# Autodesk Inventor assembly: Goniometers_70x70
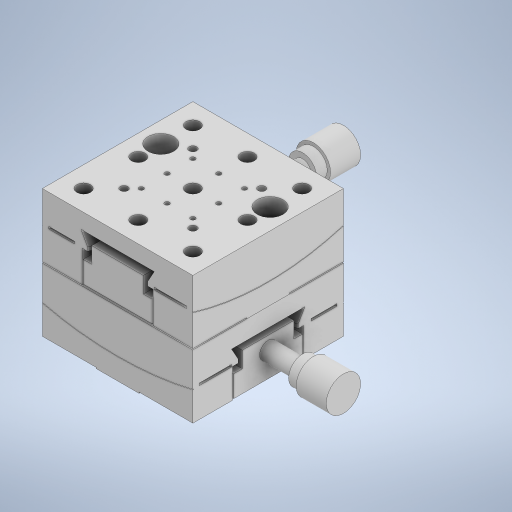
[picture p0: Inventor's stored thumbnail of the model, 512x512]
Saved by Autodesk Inventor 2024 (Build 280153000, 153)
## iProperties
Created: 2022-01-28
Part Number: Goniometers_70x70
Document SubType Name: Assembly
Designer: gnzak
Author: gnzak
## Documents named in this file (3)
- C:\Users\rosam\OneDrive\Documents\github_latest\Hardware\Tablet-Rig\Assemblies\Goniometers_70x70.iam
- C:\Users\rosam\OneDrive\Documents\github_latest\Hardware\Tablet-Rig\Parts\Edmund Optics 66-532\66532.ipt
- C:\Users\rosam\OneDrive\Documents\github_latest\Hardware\Tablet-Rig\Parts\Edmund Optics 66-533\66533.ipt
## Components (2 placed, 2 different names)
1. 66532:1 — Mate:1, Flush:1, Flush:2
2. 66533:1 — Mate:1, Flush:1, Flush:2
## Relationships (3: Flush 2, Mate 1)
- Mate:1: 66532:1 ↔ 66533:1
- Flush:1: 66532:1 ↔ 66533:1
- Flush:2: 66532:1 ↔ 66533:1
